# Autodesk Inventor assembly: MotorMountAssembly
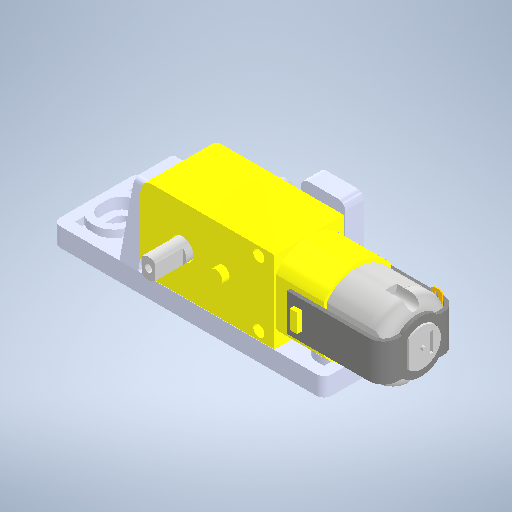
[picture p0: Inventor's stored thumbnail of the model, 512x512]
Saved by Autodesk Inventor 2026 (Build 300175050, 175E)
## iProperties
Created: 2025-06-11
Part Number: MotorMountAssembly
Document SubType Name: Assembly
Designer: omiye
Author: omiye
## Documents named in this file (3)
- C:\Projects\Arduino\strandbeest\MotorMountAssembly.iam
- C:\Projects\Arduino\strandbeest\6VDC_motor_mount_REV2.ipt
- C:\Projects\Arduino\strandbeest\yellow_toy_motor_dims.ipt
## Components (2 placed, 2 different names)
1. 6VDC_motor_mount_REV2:1 — Mate:1, Mate:2, Mate:3
2. yellow_toy_motor_dims:1 — Mate:1, Mate:2, Mate:3
## Relationships (3: Mate 3)
- Mate:1: 6VDC_motor_mount_REV2:1 ↔ yellow_toy_motor_dims:1
- Mate:2: 6VDC_motor_mount_REV2:1 ↔ yellow_toy_motor_dims:1
- Mate:3: 6VDC_motor_mount_REV2:1 ↔ yellow_toy_motor_dims:1
